# Autodesk Inventor assembly: Assemblyfull one piston111
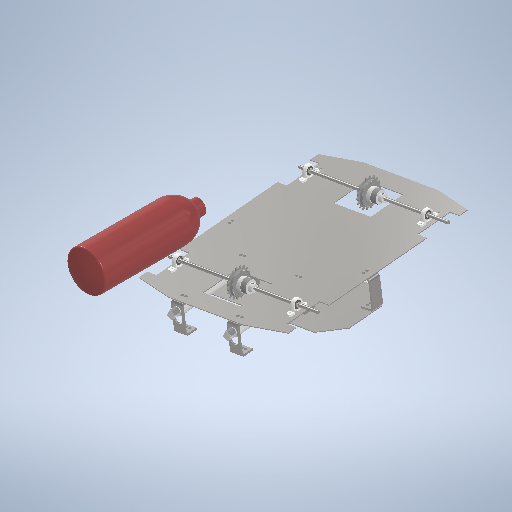
[picture p0: Inventor's stored thumbnail of the model, 512x512]
Saved by Autodesk Inventor 2026.1 (Build 301233020, 233B)
## iProperties
Created: 2026-01-22
Part Number: Assemblyfull one piston111
Document SubType Name: Assembly
Designer: user
Author: user
## Documents named in this file (11)
- D:\asu\machine element design\project\design\Assemblyfull one piston111.iam
- D:\asu\machine element design\project\design\chassis.ipt
- D:\asu\machine element design\project\design\pillow-block-bearing-p08-1.snapshot.17\Pillow Block P08\Pillow Block P08\Pillow Block P08.ipt
- D:\asu\machine element design\project\design\Assembly shaft 1 sprocect.iam
- D:\asu\machine element design\project\design\piston bracket.ipt
- D:\asu\machine element design\project\design\piston\piston .iam
- D:\asu\machine element design\project\design\tank.ipt
- D:\asu\machine element design\project\design\3dfindit-norelem-27628-08_0-0202601231542267380834410e898ce\AIS2024\27628-08_0.ipt
- C:\Users\user\Documents\Inventor\Content Center Files\R2026\en-US\ISO 4032(2)\ISO 4032 - M8 - ISO.ipt
- D:\asu\machine element design\project\design\chassis up .ipt
- D:\asu\machine element design\project\design\up bracket.ipt
## Components (21 placed, 10 different names)
1. chassis:1 — Mate:1, Mate:2, Mate:3, Mate:4, Mate:5, Mate:6, Mate:7, Mate:8, Mate:9, Mate:10, Mate:11, Mate:12, Mate:15, Mate:16, Mate:17, Mate:18, Mate:19, Mate:20, Mate:21, Mate:22, Mate:23, Mate:24, Mate:25, Mate:26, Mate:43, Mate:44, Mate:45, Mate:46, Mate:47
2. Pillow Block P08:1 — Mate:1, Mate:2, Mate:3
3. Pillow Block P08:2 — Mate:5, Mate:11, Mate:12, Mate:14
4. Pillow Block P08:3 — Mate:6, Mate:7, Mate:8
5. Pillow Block P08:4 — Mate:4, Mate:9, Mate:10, Mate:13
6. Assembly shaft 1 sprocect:1 [sub-assembly] — Mate:13
7. Assembly shaft 1 sprocect:2 [sub-assembly] — Mate:14
8. piston bracket:1 — Mate:15, Mate:17, Mate:18, Mate:39
9. piston bracket:2 — Mate:16, Mate:19, Mate:20
10. piston bracket:3 — Mate:21, Mate:22, Mate:23, Mate:29, Mate:30, Mate:41, Mate:49
11. piston bracket:4 — Mate:24, Mate:25, Mate:26, Mate:27, Mate:28, Mate:40, Mate:50
12. piston :1 [sub-assembly] — Mate:27, Mate:28, Mate:35, Mate:36, Mate:38, Mate:50
13. piston :2 [sub-assembly] — Mate:29, Mate:30, Mate:31, Mate:32, Mate:34, Mate:49
14. tank:1
15. 27628-08_0:1 — Mate:33, Mate:34
16. ISO 4032 M8:1 — Mate:31, Mate:32, Mate:33
17. ISO 4032 M8:2 — Mate:35, Mate:36, Mate:37
18. 27628-08_0:2 — Mate:37, Mate:38
19. chassis up :1 — Mate:39, Mate:40, Mate:41, Mate:42, Mate:48
20. up bracket:1 — Mate:42, Mate:43, Mate:44
21. up bracket:2 — Mate:45, Mate:46, Mate:47, Mate:48
## Relationships (50: Mate 50)
- Mate:1: chassis:1 ↔ Pillow Block P08:1
- Mate:2: chassis:1 ↔ Pillow Block P08:1
- Mate:3: chassis:1 ↔ Pillow Block P08:1
- Mate:4: chassis:1 ↔ Pillow Block P08:4
- Mate:5: chassis:1 ↔ Pillow Block P08:2
- Mate:6: chassis:1 ↔ Pillow Block P08:3
- Mate:7: chassis:1 ↔ Pillow Block P08:3
- Mate:8: chassis:1 ↔ Pillow Block P08:3
- Mate:9: chassis:1 ↔ Pillow Block P08:4
- Mate:10: chassis:1 ↔ Pillow Block P08:4
- Mate:11: chassis:1 ↔ Pillow Block P08:2
- Mate:12: chassis:1 ↔ Pillow Block P08:2
- Mate:13: Pillow Block P08:4 ↔ Assembly shaft 1 sprocect:1
- Mate:14: Pillow Block P08:2 ↔ Assembly shaft 1 sprocect:2
- Mate:15: chassis:1 ↔ piston bracket:1
- Mate:16: chassis:1 ↔ piston bracket:2
- Mate:17: chassis:1 ↔ piston bracket:1
- Mate:18: chassis:1 ↔ piston bracket:1
- Mate:19: chassis:1 ↔ piston bracket:2
- Mate:20: chassis:1 ↔ piston bracket:2
- Mate:21: chassis:1 ↔ piston bracket:3
- Mate:22: chassis:1 ↔ piston bracket:3
- Mate:23: chassis:1 ↔ piston bracket:3
- Mate:24: chassis:1 ↔ piston bracket:4
- Mate:25: chassis:1 ↔ piston bracket:4
- Mate:26: chassis:1 ↔ piston bracket:4
- Mate:27: piston bracket:4 ↔ piston :1
- Mate:28: piston bracket:4 ↔ piston :1
- Mate:29: piston bracket:3 ↔ piston :2
- Mate:30: piston bracket:3 ↔ piston :2
- Mate:31: piston :2 ↔ ISO 4032 M8:1
- Mate:32: piston :2 ↔ ISO 4032 M8:1
- Mate:33: 27628-08_0:1 ↔ ISO 4032 M8:1
- Mate:34: piston :2 ↔ 27628-08_0:1
- Mate:35: piston :1 ↔ ISO 4032 M8:2
- Mate:36: piston :1 ↔ ISO 4032 M8:2
- Mate:37: ISO 4032 M8:2 ↔ 27628-08_0:2
- Mate:38: piston :1 ↔ 27628-08_0:2
- Mate:39: piston bracket:1 ↔ chassis up :1
- Mate:40: piston bracket:4 ↔ chassis up :1
- Mate:41: piston bracket:3 ↔ chassis up :1
- Mate:42: chassis up :1 ↔ up bracket:1
- Mate:43: chassis:1 ↔ up bracket:1
- Mate:44: chassis:1 ↔ up bracket:1
- Mate:45: chassis:1 ↔ up bracket:2
- Mate:46: chassis:1 ↔ up bracket:2
- Mate:47: chassis:1 ↔ up bracket:2
- Mate:48: chassis up :1 ↔ up bracket:2
- Mate:49: piston bracket:3 ↔ piston :2
- Mate:50: piston bracket:4 ↔ piston :1
## Named parameters: sa_0 = 10000
note: some values were not read from the file. Shown as the stored number, unit unknown: "sa_0".
